# Autodesk Inventor assembly: Ankle_roll_shim_basis
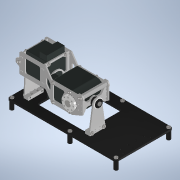
[picture p0: Inventor's stored thumbnail of the model, 180x180]
Saved by Autodesk Inventor 2020 (Build 240168000, 168)
## iProperties
Created: 2021-11-14
Part Number: Ankle_roll_shim_basis
Document SubType Name: Assembly
Designer: Masato Kubotera
Author: Masato Kubotera
## Documents named in this file (3)
- C:\Users\Masato\Documents\Inventor\CIT Brains_Inventor\OpenPlatform_ver3_0\Shim\Ankle_roll_shim_basis.iam
- C:\Users\Masato\Documents\Inventor\CIT Brains_Inventor\OpenPlatform_ver3_0\LowerBody\Foot\Foot.iam
- C:\Users\Masato\Documents\Inventor\CIT Brains_Inventor\OpenPlatform_ver3_0\LowerBody\Ankle\Ankle.iam
## Components (2 placed, 2 different names)
1. Foot:1 [sub-assembly] — 挿入:1, 角度:1
2. Ankle:1 [sub-assembly] — 挿入:1, 角度:1
## Relationships (2: Insert 1, Angle 1)
- 挿入:1 [Insert]: Foot:1 ↔ Ankle:1
- 角度:1 [Angle] (0 deg): Foot:1 ↔ Ankle:1
